# Autodesk Inventor assembly: START BUTTON
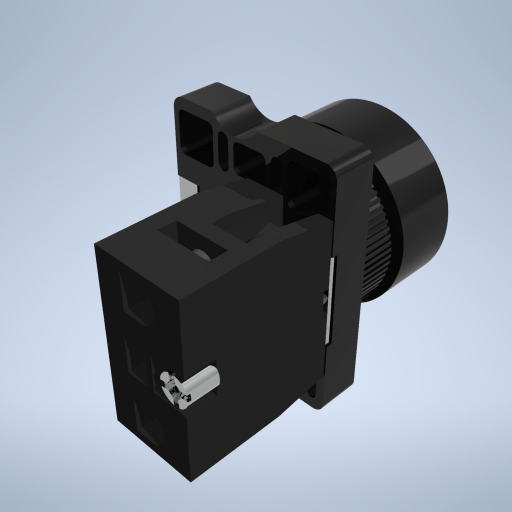
[picture p0: Inventor's stored thumbnail of the model, 512x512]
Saved by Autodesk Inventor 2023 (Build 270158000, 158)
## iProperties
Created: 2023-10-18
Part Number: START BUTTON
Document SubType Name: Assembly
Designer: vinicius.sena
Author: vinicius.sena
## Documents named in this file (10)
- C:\Users\vinicius.sena\Desktop\Vinicius\PUSH BUTTON\START BUTTON.iam
- C:\Users\vinicius.sena\Desktop\Vinicius\PUSH BUTTON\BASE.ipt
- C:\Users\vinicius.sena\Desktop\Vinicius\PUSH BUTTON\BOTÃO.ipt
- C:\Users\vinicius.sena\Desktop\Vinicius\PUSH BUTTON\CARCAÇA DO BOTÃO.ipt
- C:\Users\vinicius.sena\Desktop\Vinicius\PUSH BUTTON\PORCA DO BOTÃO.ipt
- C:\Users\vinicius.sena\Desktop\Vinicius\PUSH BUTTON\TRAVA.ipt
- C:\Users\vinicius.sena\Desktop\Vinicius\PUSH BUTTON\PARAFUSO.ipt
- C:\Users\vinicius.sena\Desktop\Vinicius\PUSH BUTTON\BLOCO DE CONTATO.ipt
- C:\Users\vinicius.sena\Desktop\Vinicius\PUSH BUTTON\PEÇA MOVEL.ipt
- C:\Users\vinicius.sena\Documents\Inventor\Content Center Files\R2023\pt-BR\CSN 02 1131  A\CSN 02 1131 - M2,5 x 3A.ipt
## Components (11 placed, 9 different names)
1. BASE:1 — Coincidente:4, Alinhado:2, Coincidente:5, Coincidente:6, Coincidente:7, Coincidente:8, Coincidente:9, Coincidente:10, Coincidente:11, Coincidente:21
2. BOTÃO:1 — Coincidente:1, Alinhado:1
3. CARCAÇA DO BOTÃO:1 — Coincidente:1, Alinhado:1, Coincidente:2, Coincidente:3, Coincidente:4, Alinhado:2, Coincidente:5
4. PORCA DO BOTÃO:1 — Coincidente:2, Coincidente:3
5. TRAVA:1 — Coincidente:9, Coincidente:10, Coincidente:11, Coincidente:12
6. TRAVA:2 — Coincidente:6, Coincidente:7, Coincidente:8
7. PARAFUSO:1 — Coincidente:13, Coincidente:14
8. BLOCO DE CONTATO:1 — Coincidente:12, Coincidente:13, Coincidente:14, Alinhado:3, Coincidente:15, Coincidente:16, Coincidente:17, Coincidente:18, Coincidente:19, Coincidente:20, Coincidente:21
9. PEÇA MOVEL:1 — Alinhado:3, Coincidente:15, Coincidente:16
10. CSN 02 1131 A M2,5 x 3:1 — Coincidente:17, Coincidente:18
11. CSN 02 1131 A M2,5 x 3:2 — Coincidente:19, Coincidente:20
## Relationships (24: Mate 21, Flush 3)
- Coincidente:1 [Mate]: BOTÃO:1 ↔ CARCAÇA DO BOTÃO:1
- Alinhado:1 [Flush]: BOTÃO:1 ↔ CARCAÇA DO BOTÃO:1
- Coincidente:2 [Mate]: CARCAÇA DO BOTÃO:1 ↔ PORCA DO BOTÃO:1
- Coincidente:3 [Mate] (1.5 mm): CARCAÇA DO BOTÃO:1 ↔ PORCA DO BOTÃO:1
- Coincidente:4 [Mate]: BASE:1 ↔ CARCAÇA DO BOTÃO:1
- Alinhado:2 [Flush]: BASE:1 ↔ CARCAÇA DO BOTÃO:1
- Coincidente:5 [Mate]: BASE:1 ↔ CARCAÇA DO BOTÃO:1
- Coincidente:6 [Mate]: BASE:1 ↔ TRAVA:2
- Coincidente:7 [Mate]: BASE:1 ↔ TRAVA:2
- Coincidente:8 [Mate]: BASE:1 ↔ TRAVA:2
- Coincidente:9 [Mate]: BASE:1 ↔ TRAVA:1
- Coincidente:10 [Mate]: BASE:1 ↔ TRAVA:1
- Coincidente:11 [Mate]: BASE:1 ↔ TRAVA:1
- Coincidente:12 [Mate]: TRAVA:1 ↔ BLOCO DE CONTATO:1
- Coincidente:13 [Mate]: PARAFUSO:1 ↔ BLOCO DE CONTATO:1
- Coincidente:14 [Mate]: PARAFUSO:1 ↔ BLOCO DE CONTATO:1
- Alinhado:3 [Flush] (3 mm): BLOCO DE CONTATO:1 ↔ PEÇA MOVEL:1
- Coincidente:15 [Mate]: BLOCO DE CONTATO:1 ↔ PEÇA MOVEL:1
- Coincidente:16 [Mate]: BLOCO DE CONTATO:1 ↔ PEÇA MOVEL:1
- Coincidente:17 [Mate]: BLOCO DE CONTATO:1 ↔ CSN 02 1131 A M2,5 x 3:1
- Coincidente:18 [Mate]: BLOCO DE CONTATO:1 ↔ CSN 02 1131 A M2,5 x 3:1
- Coincidente:19 [Mate]: BLOCO DE CONTATO:1 ↔ CSN 02 1131 A M2,5 x 3:2
- Coincidente:20 [Mate]: BLOCO DE CONTATO:1 ↔ CSN 02 1131 A M2,5 x 3:2
- Coincidente:21 [Mate]: BASE:1 ↔ BLOCO DE CONTATO:1
